# Autodesk Inventor assembly: licht_200
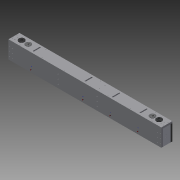
[picture p0: Inventor's stored thumbnail of the model, 180x180]
Saved by Autodesk Inventor 2015 (Build 190159000, 159)
## iProperties
Created: 2018-02-17
Part Number: licht_200
Document SubType Name: Assembly
Designer: wepet
Author: wepet
## Documents named in this file (12)
- C:\workspace\robosax\licht\Einzelteil_150\licht_150.iam
- C:\workspace\robosax\licht\Einzelteil_150\licht_150_back.ipt
- C:\workspace\robosax\licht\Einzelteil_150\licht_150_front.ipt
- C:\workspace\robosax\licht\Einzelteil_150\licht_150_top_teil.ipt
- C:\workspace\robosax\licht\Einzelteil_200\licht_200_side_middle.ipt
- C:\workspace\robosax\licht\Einzelteil_200\licht_200_support.ipt
- C:\workspace\robosax\licht\Einzelteil_200\licht_200_side_left.ipt
- C:\workspace\robosax\licht\Einzelteil_200\licht_200_side_right.ipt
- C:\workspace\robosax\licht\Zusatzelemente\licht_led_blau.ipt
- C:\workspace\robosax\licht\Zusatzelemente\licht_taster.ipt
- C:\workspace\robosax\licht\Zusatzelemente\anschluss_strom.ipt
- C:\workspace\robosax\licht\Zusatzelemente\anschluss_daten.iam
## Components (20 placed, 11 different names)
1. licht_150_back:1 — Fluchtend:3, Fluchtend:4, Fluchtend:5, Passend:9
2. licht_150_front:1 — Passend:1, Passend:2, Passend:3, Passend:4, Fluchtend:1, Fluchtend:2, Fluchtend:3, Fluchtend:4, Passend:10, Passend:13, Passend:15, Passend:18, Passend:20, Passend:21, Fluchtend:10, Passend:23, Fluchtend:11, Einfügen:1, Einfügen:2, Einfügen:3, Einfügen:4, Einfügen:5, Einfügen:6, Einfügen:7, Einfügen:8, Passend:36
3. licht_150_top_teil:1 — Passend:4, Fluchtend:1, Fluchtend:2, Fluchtend:5, Passend:8, Passend:24, Drehbar:1, Passend:26, Passend:27, Passend:28, Passend:29, Passend:30, Passend:31, Passend:32, Passend:33, Passend:34, Passend:35
4. licht_200_side_middle:1 — Passend:8, Passend:9, Passend:10, Passend:36
5. licht_200_support:1 — Passend:13, Passend:15
6. licht_200_support:2 — Passend:18, Passend:20
7. licht_200_side_left:1 — Passend:23, Passend:24, Fluchtend:11
8. licht_200_side_right:1 — Passend:21, Fluchtend:10, Passend:35
9. licht_led_blau:1 — Einfügen:4
10. licht_led_blau:2 — Einfügen:3
11. licht_led_blau:3 — Einfügen:1
12. licht_led_blau:4 — Einfügen:2
13. licht_taster:1 — Einfügen:5
14. licht_taster:2 — Einfügen:6
15. licht_taster:3 — Einfügen:7
16. licht_taster:4 — Einfügen:8
17. anschluss_strom:1 — Drehbar:1, Passend:26
18. anschluss_strom:2 — Passend:30, Passend:31
19. anschluss_daten:1 [sub-assembly] — Passend:27, Passend:28, Passend:29
20. anschluss_daten:2 [sub-assembly] — Passend:32, Passend:33, Passend:34
## Relationships (41: Mate 25, Insert 8, Flush 7, RevoluteJoint 1)
- Passend:1 [Mate]: licht_150_front:1
- Passend:2 [Mate]: licht_150_front:1
- Passend:3 [Mate]: licht_150_front:1
- Passend:4 [Mate]: licht_150_front:1 ↔ licht_150_top_teil:1
- Fluchtend:1 [Flush]: licht_150_front:1 ↔ licht_150_top_teil:1
- Fluchtend:2 [Flush]: licht_150_front:1 ↔ licht_150_top_teil:1
- Fluchtend:3 [Flush]: licht_150_back:1 ↔ licht_150_front:1
- Fluchtend:4 [Flush]: licht_150_back:1 ↔ licht_150_front:1
- Fluchtend:5 [Flush]: licht_150_back:1 ↔ licht_150_top_teil:1
- Passend:8 [Mate]: licht_150_top_teil:1 ↔ licht_200_side_middle:1
- Passend:9 [Mate]: licht_150_back:1 ↔ licht_200_side_middle:1
- Passend:10 [Mate]: licht_150_front:1 ↔ licht_200_side_middle:1
- Passend:13 [Mate]: licht_150_front:1 ↔ licht_200_support:1
- Passend:15 [Mate]: licht_150_front:1 ↔ licht_200_support:1
- Passend:18 [Mate]: licht_150_front:1 ↔ licht_200_support:2
- Passend:20 [Mate]: licht_150_front:1 ↔ licht_200_support:2
- Passend:21 [Mate]: licht_150_front:1 ↔ licht_200_side_right:1
- Fluchtend:10 [Flush]: licht_150_front:1 ↔ licht_200_side_right:1
- Passend:23 [Mate]: licht_150_front:1 ↔ licht_200_side_left:1
- Passend:24 [Mate]: licht_150_top_teil:1 ↔ licht_200_side_left:1
- Fluchtend:11 [Flush]: licht_150_front:1 ↔ licht_200_side_left:1
- Einfügen:1 [Insert] (-5 mm): licht_150_front:1 ↔ licht_led_blau:3
- Einfügen:2 [Insert] (-5 mm): licht_150_front:1 ↔ licht_led_blau:4
- Einfügen:3 [Insert]: licht_150_front:1 ↔ licht_led_blau:2
- Einfügen:4 [Insert]: licht_150_front:1 ↔ licht_led_blau:1
- Einfügen:5 [Insert] (5 mm): licht_150_front:1 ↔ licht_taster:1
- Einfügen:6 [Insert] (5 mm): licht_150_front:1 ↔ licht_taster:2
- Einfügen:7 [Insert] (5 mm): licht_150_front:1 ↔ licht_taster:3
- Einfügen:8 [Insert] (5 mm): licht_150_front:1 ↔ licht_taster:4
- Drehbar:1 [RevoluteJoint] (-7 mm): licht_150_top_teil:1 ↔ anschluss_strom:1
- Passend:26 [Mate]: licht_150_top_teil:1 ↔ anschluss_strom:1
- Passend:27 [Mate]: licht_150_top_teil:1 ↔ anschluss_daten:1
- Passend:28 [Mate]: licht_150_top_teil:1 ↔ anschluss_daten:1
- Passend:29 [Mate]: licht_150_top_teil:1 ↔ anschluss_daten:1
- Passend:30 [Mate]: licht_150_top_teil:1 ↔ anschluss_strom:2
- Passend:31 [Mate]: licht_150_top_teil:1 ↔ anschluss_strom:2
- Passend:32 [Mate]: licht_150_top_teil:1 ↔ anschluss_daten:2
- Passend:33 [Mate]: licht_150_top_teil:1 ↔ anschluss_daten:2
- Passend:34 [Mate]: licht_150_top_teil:1 ↔ anschluss_daten:2
- Passend:35 [Mate]: licht_150_top_teil:1 ↔ licht_200_side_right:1
- Passend:36 [Mate]: licht_150_front:1 ↔ licht_200_side_middle:1
